# Autodesk Inventor assembly: STM assembly
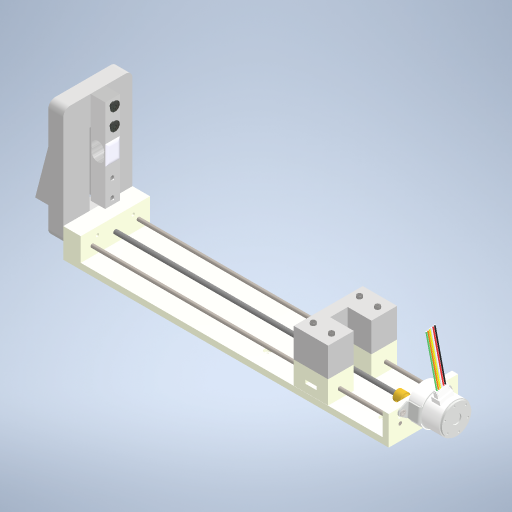
[picture p0: Inventor's stored thumbnail of the model, 512x512]
Saved by Autodesk Inventor 2024 (Build 280153000, 153)
## iProperties
Created: 2023-12-08
Part Number: STM assembly
Document SubType Name: Assembly
Designer: Abdulrahman Riskuwa
Author: Abdulrahman Riskuwa
## Documents named in this file (9)
- C:\Users\Abdulrahman Riskuwa\Documents\FMD 3 Project\STM assembly.iam
- C:\Users\Abdulrahman Riskuwa\Documents\FMD 3 Project\FMDIII.ipt
- C:\Users\Abdulrahman Riskuwa\Documents\FMD 3 Project\stand_less_rough.ipt
- C:\Users\Abdulrahman Riskuwa\Documents\Inventor\Content Center Files\R2024\en-US\ISO 4017(1)\ISO 4017 - M2 x 16 - ISO.ipt
- C:\Users\Abdulrahman Riskuwa\Documents\FMD 3 Project\shaftdrive.ipt
- C:\Users\Abdulrahman Riskuwa\Documents\FMD 3 Project\holder1.ipt
- C:\Users\Abdulrahman Riskuwa\Documents\Inventor\Content Center Files\R2024\en-US\ISO 1207(2)\ISO 1207 - M2.5 x 25.ipt
- C:\Users\Abdulrahman Riskuwa\Documents\FMD 3 Project\Weight Sensor.ipt
- C:\Users\Abdulrahman Riskuwa\Documents\Inventor\Content Center Files\R2024\en-US\ISO 10642(1)\ISO 10642 - M4 x  20.ipt
## Components (13 placed, 8 different names)
1. FMDIII:1 — Mate:1, Mate:2, Mate:7, Mate:8, Mate:9, Mate:10, Mate:11, Flush:1, Flush:2, Mate:16
2. stand_less_rough:1 — Mate:1, Mate:2, Mate:9, Mate:10, Mate:11, Mate:12, Mate:13, Mate:14, Mate:15, Mate:24
3. ISO 4017 M2 x 16:1 — Mate:12, Mate:13
4. ISO 4017 M2 x 16:2 — Mate:14, Mate:15
5. shaftdrive:1 — Mate:7, Mate:8
6. holder1:1 — Flush:1, Flush:2, Mate:17, Mate:18, Mate:19, Mate:20, Mate:21, Mate:22, Mate:23
7. ISO 1207 M2.5 x 25:1 — Mate:16, Mate:17
8. ISO 1207 M2.5 x 25:2 — Mate:18, Mate:19
9. ISO 1207 M2.5 x 25:3 — Mate:20, Mate:21
10. ISO 1207 M2.5 x 25:4 — Mate:22, Mate:23
11. Weight Sensor:1 — Mate:24, Mate:25, Mate:26, Mate:27, Mate:28
12. ISO 10642 M4x20:1 — Mate:25, Mate:26
13. ISO 10642 M4x20:2 — Mate:27, Mate:28
## Relationships (26: Mate 24, Flush 2)
- Mate:1: FMDIII:1 ↔ stand_less_rough:1
- Mate:2: FMDIII:1 ↔ stand_less_rough:1
- Mate:7: FMDIII:1 ↔ shaftdrive:1
- Mate:8: FMDIII:1 ↔ shaftdrive:1
- Mate:9: FMDIII:1 ↔ stand_less_rough:1
- Mate:10: FMDIII:1 ↔ stand_less_rough:1
- Mate:11: FMDIII:1 ↔ stand_less_rough:1
- Mate:12: stand_less_rough:1 ↔ ISO 4017 M2 x 16:1
- Mate:13: stand_less_rough:1 ↔ ISO 4017 M2 x 16:1
- Mate:14: stand_less_rough:1 ↔ ISO 4017 M2 x 16:2
- Mate:15: stand_less_rough:1 ↔ ISO 4017 M2 x 16:2
- Flush:1: FMDIII:1 ↔ holder1:1
- Flush:2: FMDIII:1 ↔ holder1:1
- Mate:16: FMDIII:1 ↔ ISO 1207 M2.5 x 25:1
- Mate:17: holder1:1 ↔ ISO 1207 M2.5 x 25:1
- Mate:18: holder1:1 ↔ ISO 1207 M2.5 x 25:2
- Mate:19: holder1:1 ↔ ISO 1207 M2.5 x 25:2
- Mate:20: holder1:1 ↔ ISO 1207 M2.5 x 25:3
- Mate:21: holder1:1 ↔ ISO 1207 M2.5 x 25:3
- Mate:22: holder1:1 ↔ ISO 1207 M2.5 x 25:4
- Mate:23: holder1:1 ↔ ISO 1207 M2.5 x 25:4
- Mate:24: stand_less_rough:1 ↔ Weight Sensor:1
- Mate:25: Weight Sensor:1 ↔ ISO 10642 M4x20:1
- Mate:26: Weight Sensor:1 ↔ ISO 10642 M4x20:1
- Mate:27: Weight Sensor:1 ↔ ISO 10642 M4x20:2
- Mate:28: Weight Sensor:1 ↔ ISO 10642 M4x20:2
